# Autodesk Inventor assembly: Ender 3 Pro Assembly
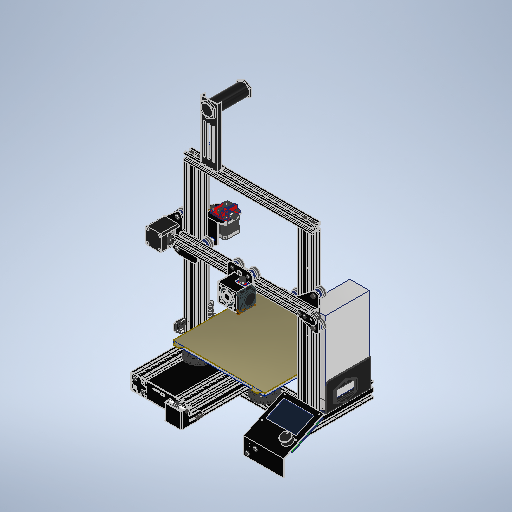
[picture p0: Inventor's stored thumbnail of the model, 512x512]
Saved by Autodesk Inventor 2025 (Build 290162000, 162)
## iProperties
Created: 2025-04-09
Part Number: Ender 3 Pro Assembly
Document SubType Name: Assembly
Designer: MAL16204
Author: MAL16204
## Documents named in this file (89)
- C:\Users\MAL16204\OneDrive - Pennsylvania Western University\Spring 2025\MECH 2400\CAD Projects\Final Project\Ender 3 Pro Assembly.iam
- C:\Users\MAL16204\OneDrive - Pennsylvania Western University\Spring 2025\MECH 2400\CAD Projects\Final Project\Aluminum Extrusions\4040 Central Profile.ipt
- C:\Users\MAL16204\OneDrive - Pennsylvania Western University\Spring 2025\MECH 2400\CAD Projects\Final Project\Aluminum Extrusions\4040 Left Profile.ipt
- C:\Users\MAL16204\OneDrive - Pennsylvania Western University\Spring 2025\MECH 2400\CAD Projects\Final Project\Aluminum Extrusions\4040 Right Profile.ipt
- C:\Users\MAL16204\OneDrive - Pennsylvania Western University\Spring 2025\MECH 2400\CAD Projects\Final Project\Aluminum Extrusions\2040 Right Profile.ipt
- C:\Users\MAL16204\OneDrive - Pennsylvania Western University\Spring 2025\MECH 2400\CAD Projects\Final Project\Aluminum Extrusions\2040 Left Profile.ipt
- C:\Users\MAL16204\OneDrive - Pennsylvania Western University\Spring 2025\MECH 2400\CAD Projects\Final Project\Aluminum Extrusions\2020 Top Profile.ipt
- C:\Users\MAL16204\OneDrive - Pennsylvania Western University\Spring 2025\MECH 2400\CAD Projects\Final Project\Miscellaneous Hardware\BS EN ISO 4762 - M5 x 50(1).ipt
- C:\Users\MAL16204\OneDrive - Pennsylvania Western University\Spring 2025\MECH 2400\CAD Projects\Final Project\Filament Holder\Support Frame (Filament Holder.ipt
- C:\Users\MAL16204\OneDrive - Pennsylvania Western University\Spring 2025\MECH 2400\CAD Projects\Final Project\Filament Holder\Support Tube (Filament Holder.ipt
- C:\Users\MAL16204\OneDrive - Pennsylvania Western University\Spring 2025\MECH 2400\CAD Projects\Final Project\Filament Holder\M30 Plastic Nut.ipt
- C:\Users\MAL16204\OneDrive - Pennsylvania Western University\Spring 2025\MECH 2400\CAD Projects\Final Project\Aluminum Extrusions\2020 X Profile.ipt
- C:\Users\MAL16204\OneDrive - Pennsylvania Western University\Spring 2025\MECH 2400\CAD Projects\Final Project\X-Axis Supporting Cast\X Adjustment Block.ipt
- C:\Users\MAL16204\OneDrive - Pennsylvania Western University\Spring 2025\MECH 2400\CAD Projects\Final Project\X-Axis Supporting Cast\X Motor Bracket.ipt
- C:\Users\MAL16204\OneDrive - Pennsylvania Western University\Spring 2025\MECH 2400\CAD Projects\Final Project\Stepper Motor 42mm\Assembly1.iam
- C:\Users\MAL16204\OneDrive - Pennsylvania Western University\Spring 2025\MECH 2400\CAD Projects\Final Project\Miscellaneous Hardware\Spacers for Rollers.ipt
- C:\Users\MAL16204\OneDrive - Pennsylvania Western University\Spring 2025\MECH 2400\CAD Projects\Final Project\Miscellaneous Hardware\Wheel_24.4mm v1\Wheel_24.4mm v1.ipt
- C:\Users\MAL16204\OneDrive - Pennsylvania Western University\Spring 2025\MECH 2400\CAD Projects\Final Project\Extruder\E Motor Bracket.ipt
- C:\Users\MAL16204\OneDrive - Pennsylvania Western University\Spring 2025\MECH 2400\CAD Projects\Final Project\LCD Support\LCD Support.ipt
- C:\Users\MAL16204\OneDrive - Pennsylvania Western University\Spring 2025\MECH 2400\CAD Projects\Final Project\LCD Support\LCD Knob.ipt
- C:\Users\MAL16204\OneDrive - Pennsylvania Western University\Spring 2025\MECH 2400\CAD Projects\Final Project\Aluminum Extrusions\4040 Y Profile.ipt
- C:\Users\MAL16204\OneDrive - Pennsylvania Western University\Spring 2025\MECH 2400\CAD Projects\Final Project\Z-Axis Supporting Cast\Z Stent.ipt
- C:\Users\MAL16204\OneDrive - Pennsylvania Western University\Spring 2025\MECH 2400\CAD Projects\Final Project\Hotend Assembly\Workspaces\Workspace\Extruder Plate.ipt
- C:\Users\MAL16204\OneDrive - Pennsylvania Western University\Spring 2025\MECH 2400\CAD Projects\Final Project\Hotend Assembly\Workspaces\Workspace\Hotend.ipt
- C:\Users\MAL16204\OneDrive - Pennsylvania Western University\Spring 2025\MECH 2400\CAD Projects\Final Project\Hotend Assembly\Workspaces\Workspace\Nozzle 0.4mm.ipt
- C:\Users\MAL16204\OneDrive - Pennsylvania Western University\Spring 2025\MECH 2400\CAD Projects\Final Project\Hotend Assembly\Workspaces\Workspace\Fan Cover.ipt
- C:\Users\MAL16204\OneDrive - Pennsylvania Western University\Spring 2025\MECH 2400\CAD Projects\Final Project\Y-Axis Supporting Cast\Y plate(GITHUB CR)\Y plate(GITHUB CR)\Y plate(GITHUB CR).ipt
- C:\Users\MAL16204\OneDrive - Pennsylvania Western University\Spring 2025\MECH 2400\CAD Projects\Final Project\Y-Axis Supporting Cast\Build Plate.ipt
- C:\Users\MAL16204\OneDrive - Pennsylvania Western University\Spring 2025\MECH 2400\CAD Projects\Final Project\Y-Axis Supporting Cast\Build Plate Rubber Supports.ipt
- C:\Users\MAL16204\OneDrive - Pennsylvania Western University\Spring 2025\MECH 2400\CAD Projects\Final Project\Z-Axis Supporting Cast\Z Nut.ipt
- C:\Users\MAL16204\OneDrive - Pennsylvania Western University\Spring 2025\MECH 2400\CAD Projects\Final Project\Sheetmetal Enclosures\Sheetmetal Enclosure Top.ipt
- C:\Users\MAL16204\OneDrive - Pennsylvania Western University\Spring 2025\MECH 2400\CAD Projects\Final Project\Sheetmetal Enclosures\Sheetmetal Enclosure Bottom.ipt
- C:\Users\MAL16204\OneDrive - Pennsylvania Western University\Spring 2025\MECH 2400\CAD Projects\Final Project\Y-Axis Supporting Cast\PEI Sheet (Build Plate).ipt
- C:\Users\MAL16204\OneDrive - Pennsylvania Western University\Spring 2025\MECH 2400\CAD Projects\Final Project\Y-Axis Supporting Cast\Hand Twisted Nut\Hand Twisted Nut\Hand Twisted Nut.ipt
- C:\Users\MAL16204\OneDrive - Pennsylvania Western University\Spring 2025\MECH 2400\CAD Projects\Final Project\Z-Axis Supporting Cast\Z Axis Motor Mount.ipt
- C:\Users\MAL16204\OneDrive - Pennsylvania Western University\Spring 2025\MECH 2400\CAD Projects\Final Project\Z-Axis Supporting Cast\Lead Screw Holder.ipt
- C:\Users\MAL16204\OneDrive - Pennsylvania Western University\Spring 2025\MECH 2400\CAD Projects\Final Project\Extruder\E housing\E housing.ipt
- C:\Users\MAL16204\OneDrive - Pennsylvania Western University\Spring 2025\MECH 2400\CAD Projects\Final Project\Extruder\E gear\E gear.ipt
- C:\Users\MAL16204\OneDrive - Pennsylvania Western University\Spring 2025\MECH 2400\CAD Projects\Final Project\Extruder\E idler tensioner\E idler tensioner.ipt
- C:\Users\MAL16204\OneDrive - Pennsylvania Western University\Spring 2025\MECH 2400\CAD Projects\Final Project\Z-Axis Supporting Cast\Lead Screw.ipt
- C:\Users\MAL16204\OneDrive - Pennsylvania Western University\Spring 2025\MECH 2400\CAD Projects\Final Project\LCD Support\lcd\lcd\lcd.ipt
- C:\Users\MAL16204\OneDrive - Pennsylvania Western University\Spring 2025\MECH 2400\CAD Projects\Final Project\Extruder\Extrusion Spring\Extrusion Spring\Extrusion Spring.ipt
- C:\Users\MAL16204\OneDrive - Pennsylvania Western University\Spring 2025\MECH 2400\CAD Projects\Final Project\Extruder\Pneumatic joint\Pneumatic joint\Pneumatic joint.ipt
- C:\Users\MAL16204\OneDrive - Pennsylvania Western University\Spring 2025\MECH 2400\CAD Projects\Final Project\Content Center Files\en-US\en-US\ISO 7380-1\ISO 7380-1 - M5 x 35.ipt
- C:\Users\MAL16204\OneDrive - Pennsylvania Western University\Spring 2025\MECH 2400\CAD Projects\Final Project\Content Center Files\en-US\en-US\ISO 7380-1\ISO 7380-1 - M5 x 25.ipt
- C:\Users\MAL16204\OneDrive - Pennsylvania Western University\Spring 2025\MECH 2400\CAD Projects\Final Project\Content Center Files\en-US\en-US\ISO 7380-1\ISO 7380-1 - M4 x 25.ipt
- C:\Users\MAL16204\OneDrive - Pennsylvania Western University\Spring 2025\MECH 2400\CAD Projects\Final Project\Power Supply\Power holder\Power holder\Power holder.ipt
- C:\Users\MAL16204\OneDrive - Pennsylvania Western University\Spring 2025\MECH 2400\CAD Projects\Final Project\Power Supply\24V15A power supply\24V15A power supply\24V15A power supply.ipt
- C:\Users\MAL16204\OneDrive - Pennsylvania Western University\Spring 2025\MECH 2400\CAD Projects\Final Project\Content Center Files\en-US\ISO 7380-1\ISO 7380-1 - M5 x 8.ipt
- C:\Users\MAL16204\OneDrive - Pennsylvania Western University\Spring 2025\MECH 2400\CAD Projects\Final Project\Content Center Files\en-US\ISO 7380-1\ISO 7380-1 - M4 x 6.ipt
- C:\Users\MAL16204\OneDrive - Pennsylvania Western University\Spring 2025\MECH 2400\CAD Projects\Final Project\Content Center Files\en-US\ISO 7380-1\ISO 7380-1 - M3 x 6.ipt
- C:\Users\MAL16204\OneDrive - Pennsylvania Western University\Spring 2025\MECH 2400\CAD Projects\Final Project\Content Center Files\en-US\BS EN ISO 4762\BS EN ISO 4762 - M2.5 x 4(1).ipt
- C:\Users\MAL16204\OneDrive - Pennsylvania Western University\Spring 2025\MECH 2400\CAD Projects\Final Project\Content Center Files\en-US\BS 4168(8)\BS 4168 - M4 x 25(7).ipt
- C:\Users\MAL16204\OneDrive - Pennsylvania Western University\Spring 2025\MECH 2400\CAD Projects\Final Project\Content Center Files\en-US\BS 4168(8)\BS 4168 - M3 x 16(7).ipt
- C:\Users\MAL16204\OneDrive - Pennsylvania Western University\Spring 2025\MECH 2400\CAD Projects\Final Project\Content Center Files\en-US\ISO 7380-1\ISO 7380-1 - M3 x 10.ipt
- C:\Users\MAL16204\OneDrive - Pennsylvania Western University\Spring 2025\MECH 2400\CAD Projects\Final Project\Content Center Files\en-US\ISO 4032(2)\ISO 4032 - M4 - ISO.ipt
- C:\Users\MAL16204\OneDrive - Pennsylvania Western University\Spring 2025\MECH 2400\CAD Projects\Final Project\Content Center Files\en-US\ISO 4032(2)\ISO 4032 - M5 - ISO.ipt
- C:\Users\MAL16204\OneDrive - Pennsylvania Western University\Spring 2025\MECH 2400\CAD Projects\Final Project\Miscellaneous Hardware\TSlot Nut.ipt
- C:\Users\MAL16204\OneDrive - Pennsylvania Western University\Spring 2025\MECH 2400\CAD Projects\Final Project\Content Center Files\en-US\ISO 7380-1\ISO 7380-1 - M5 x 10.ipt
- C:\Users\MAL16204\OneDrive - Pennsylvania Western University\Spring 2025\MECH 2400\CAD Projects\Final Project\Content Center Files\en-US\ISO 7380-1\ISO 7380-1 - M4 x 8.ipt
- C:\Users\MAL16204\OneDrive - Pennsylvania Western University\Spring 2025\MECH 2400\CAD Projects\Final Project\Content Center Files\en-US\ISO 7380-1\ISO 7380-1 - M5 x 12.ipt
- C:\Users\MAL16204\OneDrive - Pennsylvania Western University\Spring 2025\MECH 2400\CAD Projects\Final Project\Content Center Files\en-US\ISO 7380-1\ISO 7380-1 - M4 x 16.ipt
- C:\Users\MAL16204\OneDrive - Pennsylvania Western University\Spring 2025\MECH 2400\CAD Projects\Final Project\Content Center Files\en-US\BS EN ISO 4762\BS EN ISO 4762 - M3 x 12(1).ipt
- C:\Users\MAL16204\OneDrive - Pennsylvania Western University\Spring 2025\MECH 2400\CAD Projects\Final Project\Y-Axis Supporting Cast\Y Belt Adjuster.ipt
- C:\Users\MAL16204\OneDrive - Pennsylvania Western University\Spring 2025\MECH 2400\CAD Projects\Final Project\Y-Axis Supporting Cast\Roller Spacers.ipt
- C:\Users\MAL16204\OneDrive - Pennsylvania Western University\Spring 2025\MECH 2400\CAD Projects\Final Project\Y-Axis Supporting Cast\Belt Tension Rollers.ipt
- C:\Users\MAL16204\OneDrive - Pennsylvania Western University\Spring 2025\MECH 2400\CAD Projects\Final Project\Content Center Files\en-US\ISO 4762(2)\ISO 4762 - M3 x 30ISO.ipt
- C:\Users\MAL16204\OneDrive - Pennsylvania Western University\Spring 2025\MECH 2400\CAD Projects\Final Project\Content Center Files\en-US\ISO 4032(2)\ISO 4032 - M3.5 - ISO.ipt
- C:\Users\MAL16204\OneDrive - Pennsylvania Western University\Spring 2025\MECH 2400\CAD Projects\Final Project\Content Center Files\en-US\BS EN ISO 4762\BS EN ISO 4762 - M4 x 40(1).ipt
- C:\Users\MAL16204\OneDrive - Pennsylvania Western University\Spring 2025\MECH 2400\CAD Projects\Final Project\Content Center Files\en-US\ISO 7380-1\ISO 7380-1 - M3 x 16.ipt
- C:\Users\MAL16204\OneDrive - Pennsylvania Western University\Spring 2025\MECH 2400\CAD Projects\Final Project\Hotend Assembly\Nozzle fan\Nozzle fan\Nozzle fan.ipt
- C:\Users\MAL16204\OneDrive - Pennsylvania Western University\Spring 2025\MECH 2400\CAD Projects\Final Project\Content Center Files\en-US\BS EN ISO 4762\BS EN ISO 4762 - M3 x 8(1).ipt
- C:\Users\MAL16204\OneDrive - Pennsylvania Western University\Spring 2025\MECH 2400\CAD Projects\Final Project\Hotend Assembly\Nozzle fan duct\Nozzle fan duct\Nozzle fan duct.ipt
- C:\Users\MAL16204\OneDrive - Pennsylvania Western University\Spring 2025\MECH 2400\CAD Projects\Final Project\Hotend Assembly\Cold section fan\Cold section fan\Cold section fan.ipt
- C:\Users\MAL16204\OneDrive - Pennsylvania Western University\Spring 2025\MECH 2400\CAD Projects\Final Project\Y-Axis Supporting Cast\Y Motor Bracket.ipt
- C:\Users\MAL16204\OneDrive - Pennsylvania Western University\Spring 2025\MECH 2400\CAD Projects\Final Project\Y-Axis Supporting Cast\Y Limit Switch Bracket.ipt
- C:\Users\MAL16204\OneDrive - Pennsylvania Western University\Spring 2025\MECH 2400\CAD Projects\Final Project\Y-Axis Supporting Cast\limit switch\limit switch\limit switch.ipt
- C:\Users\MAL16204\OneDrive - Pennsylvania Western University\Spring 2025\MECH 2400\CAD Projects\Final Project\Content Center Files\en-US\ISO 7380-1\ISO 7380-1 - M4 x 10.ipt
- C:\Users\MAL16204\OneDrive - Pennsylvania Western University\Spring 2025\MECH 2400\CAD Projects\Final Project\Z-Axis Supporting Cast\Z Limit Switch Bracket.ipt
- C:\Users\MAL16204\OneDrive - Pennsylvania Western University\Spring 2025\MECH 2400\CAD Projects\Final Project\Content Center Files\en-US\ISO 7380-1\ISO 7380-1 - M4 x 30.ipt
- C:\Users\MAL16204\OneDrive - Pennsylvania Western University\Spring 2025\MECH 2400\CAD Projects\Final Project\Miscellaneous Hardware\Eccentric Column.ipt
- C:\Users\MAL16204\OneDrive - Pennsylvania Western University\Spring 2025\MECH 2400\CAD Projects\Final Project\Content Center Files\en-US\ISO 10642(1)\ISO 10642 - M3 x  20.ipt
- C:\Users\MAL16204\OneDrive - Pennsylvania Western University\Spring 2025\MECH 2400\CAD Projects\Final Project\Content Center Files\en-US\ISO 4026\ISO 4026 - M3 x 5 - ISO.ipt
- C:\Users\MAL16204\OneDrive - Pennsylvania Western University\Spring 2025\MECH 2400\CAD Projects\Final Project\Content Center Files\en-US\ISO 104\ISO 104 - 0 70 - 4 x 12 x 4.ipt
- C:\Users\MAL16204\OneDrive - Pennsylvania Western University\Spring 2025\MECH 2400\CAD Projects\Final Project\Content Center Files\en-US\BS EN ISO 4762\BS EN ISO 4762 - M3 x 6(1).ipt
- C:\Users\MAL16204\OneDrive - Pennsylvania Western University\Spring 2025\MECH 2400\CAD Projects\Final Project\X-Axis Supporting Cast\XEndStopHolder.ipt
- C:\Users\MAL16204\OneDrive - Pennsylvania Western University\Spring 2025\MECH 2400\CAD Projects\Final Project\Content Center Files\en-US\BS EN ISO 4762\BS EN ISO 4762 - M4 x 25(1).ipt
- C:\Users\MAL16204\OneDrive - Pennsylvania Western University\Spring 2025\MECH 2400\CAD Projects\Final Project\Content Center Files\en-US\ISO 4762(2)\ISO 4762 - M2 x 3ISO.ipt
- C:\Users\MAL16204\OneDrive - Pennsylvania Western University\Spring 2025\MECH 2400\CAD Projects\Final Project\Content Center Files\en-US\ISO 7380-1\ISO 7380-1 - M3 x 8.ipt
## Components (217 placed, 88 different names)
1. 4040 Central Profile:1 — Flush:1, Mate:1, Mate:2, Flush:2, Mate:3, Mate:4, Flush:4, Mate:21, Mate:22, Flush:11, Mate:39
2. 4040 Left Profile:1 — Flush:1, Mate:1, Mate:2, Mate:8, Flush:3, Rigid:2, Rigid:3, Rigid:4, Rigid:5, Mate:38, Flush:35, Flush:39, Mate:52, Mate:172
3. 4040 Right Profile:1 — Flush:2, Mate:3, Mate:4, Mate:5, Mate:6, Mate:7, Rigid:1, Cylindrical:1, Rigid:6, Rotational:1, Rigid:20, Mate:87, Flush:46
4. 2040 Right Profile:1 — Mate:5, Mate:6, Mate:7, Flush:5, Mate:24, Mate:25, Mate:26, Mate:88
5. 2040 Left Profile:1 — Mate:8, Flush:3, Flush:4, Mate:9, Flush:6, Flush:9, Mate:13, Mate:47, Mate:48, Mate:49, Mate:50, Mate:171, Flush:50, Mate:176, Mate:177, Mate:178, Mate:179
6. 2020 Top Profile:1 — Mate:9, Flush:5, Flush:6, Rigid:7, Rigid:8, Rigid:9, Rigid:10, Mate:10, Flush:7, Flush:8, Mate:115, Mate:116, Mate:118, Mate:119
7. BS EN ISO 4762 - Metric M5 x 50:1 — Rigid:1
8. BS EN ISO 4762 - Metric M5 x 50:2 — Cylindrical:1
9. BS EN ISO 4762 - Metric M5 x 50:3 — Rigid:3
10. BS EN ISO 4762 - Metric M5 x 50:4 — Rigid:2
11. BS EN ISO 4762 - Metric M5 x 50:5 — Rigid:5
12. BS EN ISO 4762 - Metric M5 x 50:6 — Rigid:4
13. BS EN ISO 4762 - Metric M5 x 50:7 — Rigid:6
14. BS EN ISO 4762 - Metric M5 x 50:8 — Rotational:1
15. BS EN ISO 4762 - Metric M5 x 50:9 — Rigid:8
16. BS EN ISO 4762 - Metric M5 x 50:10 — Rigid:7
17. BS EN ISO 4762 - Metric M5 x 50:11 — Rigid:9
18. BS EN ISO 4762 - Metric M5 x 50:12 — Rigid:10
19. Support Frame (Filament Holder:1 — Mate:10, Flush:7, Flush:8, Mate:117, Mate:120, Insert:27, Insert:28, Rigid:75
20. Support Tube (Filament Holder:1 — Rigid:11, Rigid:75, Rigid:76
21. M30 Plastic Nut:1 — Rigid:11
22. X Motor Bracket:1 — Mate:52, Rigid:61, Rigid:62, Mate:55, Mate:56, Mate:57, Rigid:63, Mate:71, Mate:72, Mate:73, Mate:74, Mate:81, Mate:82, Rigid:70, Insert:33, Insert:34, Mate:197, Mate:198, Mate:207
23. Spacers for Rollers:1 — Rotational:5, Rigid:62
24. Spacers for Rollers:2 — Rotational:3, Rigid:61
25. Spacers for Rollers:3 — Rotational:4, Rigid:63
26. Wheel_24.4mm v1:1 — Rotational:4, Rigid:16
27. Wheel_24.4mm v1:2 — Rotational:3, Rigid:17
28. Wheel_24.4mm v1:3 — Rotational:5, Flush:9, Mate:13, Rigid:15
29. E Motor Bracket:1 — Rigid:18, Rigid:19, Mate:35, Mate:36, Mate:37, Mate:58, Mate:59, Mate:64, Rotation/Translation:1, Mate:65, Mate:104, Mate:106, Mate:108, Mate:208, Mate:210
30. Spacers for Rollers:4 — Rigid:15, Rigid:19
31. Spacers for Rollers:5 — Rigid:16
32. Spacers for Rollers:6 — Rigid:17, Rigid:18
33. X Adjustment Block:1 — Mate:84, Flush:45, Mate:121, Mate:124, Mate:127, Insert:30, Insert:31, Mate:148, Mate:149
34. LCD Support:1 — Rigid:20, Rotational:6, Insert:6, Insert:7, Rigid:73
35. LCD Knob:1 — Rotational:6
36. 4040 Y Profile:1 — Mate:21, Mate:22, Flush:11, Rigid:21, Rigid:22, Rigid:23, Rigid:24, Flush:33, Flush:34, Mate:31, Mate:136, Flush:47, Mate:137, Mate:139, Mate:141, Mate:156, Mate:157, Mate:158, Mate:164, Mate:165, Mate:166, Mate:168, Mate:169, Flush:49
37. BS EN ISO 4762 - Metric M5 x 50:13 — Rigid:21
38. BS EN ISO 4762 - Metric M5 x 50:14 — Rigid:22
39. BS EN ISO 4762 - Metric M5 x 50:15 — Rigid:23
40. BS EN ISO 4762 - Metric M5 x 50:16 — Rigid:24
41. Z Stent:1 — Rigid:26, Rigid:27, Rigid:28, Flush:44, Mate:83, Rigid:72, Mate:110, Mate:112, Insert:29, Insert:32
42. Spacers for Rollers:8 — Rigid:26, Mate:28, Rigid:67
43. Spacers for Rollers:9 — Rigid:27, Mate:27
44. Spacers for Rollers:10 — Rigid:28, Mate:29
45. Wheel_24.4mm v1:4 — Mate:25, Mate:29, Mate:114
46. Wheel_24.4mm v1:5 — Mate:26, Mate:28, Rigid:67, Rigid:68
47. Wheel_24.4mm v1:6 — Mate:24, Mate:27, Rigid:69
48. Extruder Plate:1 — Rigid:29, Rigid:31, Rigid:35, Rigid:37, Insert:3, Insert:4, Flush:43, Rigid:82, Mate:190, Mate:192
49. Wheel_24.4mm v1:7 — Rigid:81, Rigid:84
50. Wheel_24.4mm v1:8 — Rigid:33, Mate:78, Mate:98
51. Wheel_24.4mm v1:9 — Rigid:34, Mate:77, Mate:100
52. Spacers for Rollers:11 — Rigid:29, Rigid:34
53. Spacers for Rollers:13 — Rigid:31, Rigid:33
54. Hotend:1 — Rigid:35, Rigid:36, Rigid:66, Mate:186, Mate:187, Mate:188, Mate:189, Flush:51
55. Nozzle 0.4mm:1 — Rigid:36
56. Fan Cover:1 — Rigid:37, Rigid:74, Mate:150, Mate:151, Mate:152, Mate:153, Mate:154, Mate:155, Mate:191, Mate:193, Mate:212, Mate:218, Mate:220, Mate:222
57. Spacers for Rollers:14 — Rigid:43, Rigid:46
58. Spacers for Rollers:15 — Rigid:44, Rigid:45
59. Wheel_24.4mm v1:12 — Rigid:43, Insert:57
60. Wheel_24.4mm v1:13 — Rigid:44, Flush:34, Insert:58
61. Y plate(GITHUB CR):1 — Rigid:45, Rigid:46, Flush:33, Mate:31, Mate:32, Mate:33, Mate:34, Mate:183, Mate:185, Rigid:78, Rigid:80
62. Wheel_24.4mm v1:15 — Rigid:77
63. Build Plate:1 — Rigid:51, Rigid:52, Rigid:53, Rigid:54, Mate:33, Mate:34, Mate:42, Flush:37, Flush:38, Rigid:56, Rigid:57, Rigid:58, Rigid:59
64. Build Plate Rubber Supports:1 — Rigid:51, Mate:32
65. Build Plate Rubber Supports:2 — Rigid:52
66. Build Plate Rubber Supports:3 — Rigid:54
67. Build Plate Rubber Supports:4 — Rigid:53
68. Assembly1:2 [sub-assembly] — Mate:35, Mate:36, Mate:37, Mate:60, Rotational:62
69. Sheetmetal Enclosure Top:1 — Mate:38, Mate:39, Flush:35, Mate:40, Mate:41, Flush:36, Insert:8, Insert:9
70. Sheetmetal Enclosure Bottom:1 — Mate:40, Mate:41, Flush:36, Insert:59, Insert:60
71. PEI Sheet (Build Plate):1 — Mate:42, Flush:37, Flush:38, Mate:80
72. Hand Twisted Nut:1 — Rigid:59
73. Hand Twisted Nut:2 — Rigid:56
74. Hand Twisted Nut:3 — Rigid:58
75. Hand Twisted Nut:4 — Rigid:57
76. Assembly1:3 [sub-assembly] — Mate:47, Flush:39, Mate:51, Rotational:61
77. Z Axis Motor Mount:1 — Mate:48, Mate:49, Mate:50, Mate:51, Mate:94, Mate:95, Insert:16, Insert:17
78. Lead Screw Holder:1 — Rotational:61, Rigid:64, Rotation/Translation:1, Insert:14, Insert:15
79. Assembly1:4 [sub-assembly] — Mate:55, Mate:56, Mate:57
80. E housing:1 — Mate:58, Mate:59, Mate:60, Rigid:65, Mate:68, Mate:69, Mate:70, Rigid:71, Mate:96, Insert:18, Insert:20
81. E gear:1 — Rotational:62
82. E idler tensioner:1 — Rigid:65, Insert:35, Insert:61
83. Lead Screw:1 — Rigid:64, Mate:63
84. Z Nut:1 — Mate:63, Mate:64, Mate:65, Mate:209, Mate:211
85. lcd:1 — Rigid:73, Insert:23, Insert:24, Insert:25, Insert:26
86. Extrusion Spring:1 — Mate:68, Mate:69, Mate:70
87. Pneumatic joint:2 — Rigid:66
88. ISO 7380-1 M5 x 35:1 — Mate:71, Mate:72, Mate:107
89. ISO 7380-1 M5 x 35:2 — Mate:73, Mate:74, Mate:105
90. ISO 7380-1 M4 x 25:1 — Insert:3, Mate:99
91. ISO 7380-1 M4 x 25:2 — Insert:4, Mate:97
92. 2020 X Profile:1 — Flush:43, Mate:77, Mate:78, Mate:80, Mate:81, Mate:82, Flush:44, Mate:83, Mate:84, Flush:45, Mate:121, Mate:122, Mate:123, Mate:125, Mate:126
93. ISO 7380-1 M5 x 25:4 — Rigid:68, Mate:109
94. ISO 7380-1 M5 x 25:5 — Rigid:69, Mate:111
95. ISO 7380-1 M5 x 35:3 — Rigid:70, Mate:103
96. Power holder:1 — Mate:87, Mate:88, Flush:46, Mate:89, Mate:90, Mate:91
97. 24V15A power supply:1 — Mate:89, Mate:90, Mate:91
98. Pneumatic joint:3 — Rigid:71
99. ISO 7380-1 M5 x 8:1 — Insert:6
100. ISO 7380-1 M5 x 8:2 — Insert:7
101. ISO 7380-1 M4 x 6:1 — Insert:8
102. ISO 7380-1 M4 x 6:2 — Insert:9
103. BS EN ISO 4762 - Metric M2.5 x 4:1 — Insert:14
104. BS EN ISO 4762 - Metric M2.5 x 4:2 — Insert:15
105. BS 4168 : Part 8 Hexagon socket countersunk and button head screws - Metric series - Metric M4 x 25:1 — Mate:94
106. BS 4168 : Part 8 Hexagon socket countersunk and button head screws - Metric series - Metric M4 x 25:2 — Mate:95
107. ISO 7380-1 M3 x 6:5 — Insert:16
108. ISO 7380-1 M3 x 6:6 — Insert:17
109. BS 4168 : Part 8 Hexagon socket countersunk and button head screws - Metric series - Metric M3 x 16:1 — Mate:96
110. ISO 7380-1 M3 x 6:7 — Insert:18
111. ISO 7380-1 M3 x 6:9 — Insert:20
112. ISO 7380-1 M4 x 25:3 — Rigid:72, Mate:113
113. ISO 7380-1 M3 x 10:1 — Insert:23
114. ISO 7380-1 M3 x 10:2 — Insert:24
115. ISO 7380-1 M3 x 10:3 — Insert:25
116. ISO 7380-1 M3 x 10:4 — Insert:26
117. ISO 4032 M4:1 — Mate:97, Mate:98
118. ISO 4032 M4:2 — Mate:99, Mate:100
119. ISO 4032 M5:2 — Mate:103, Mate:104
120. ISO 4032 M5:3 — Mate:105, Mate:106
121. ISO 4032 M5:4 — Mate:107, Mate:108
122. ISO 4032 M5:5 — Mate:109, Mate:110
123. ISO 4032 M5:6 — Mate:111, Mate:112
124. ISO 4032 M4:3 — Mate:113, Mate:114
125. TSlot Nut:1 — Mate:115, Mate:116, Mate:117
126. TSlot Nut:2 — Mate:118, Mate:119, Mate:120
127. ISO 7380-1 M5 x 8:3 — Insert:27
128. ISO 7380-1 M5 x 8:4 — Insert:28
129. ISO 7380-1 M5 x 10:1 — Insert:29
130. TSlot Nut:4 — Mate:122, Mate:123, Mate:124
131. TSlot Nut:5 — Mate:125, Mate:126, Mate:127
132. ISO 7380-1 M4 x 8:1 — Insert:30
133. ISO 7380-1 M4 x 8:2 — Insert:31
134. ISO 7380-1 M5 x 12:1 — Insert:32
135. ISO 7380-1 M4 x 16:1 — Insert:33
136. ISO 7380-1 M4 x 16:2 — Insert:34
137. BS EN ISO 4762 - Metric M3 x 12:1 — Insert:35
138. Y Belt Adjuster:1 — Mate:128, Mate:129, Mate:130, Mate:131, Insert:36, Insert:37, Mate:136, Flush:47, Mate:137, Mate:138, Mate:140, Mate:143, Mate:145
139. Roller Spacers:1 — Mate:128, Mate:129, Mate:134, Mate:135
140. Roller Spacers:2 — Mate:130, Mate:131
141. Belt Tension Rollers:1 — Mate:132, Mate:133, Mate:135
142. Belt Tension Rollers:2 — Mate:132, Mate:133, Mate:134
143. ISO 4762 M3 x 30:1 — Insert:36
144. ISO 4032 M3.5:1 — Insert:37
145. BS EN ISO 4762 - Metric M4 x 40:1 — Mate:138, Mate:139, Mate:144
146. BS EN ISO 4762 - Metric M4 x 40:2 — Mate:140, Mate:141, Mate:142
147. ISO 4032 M4:4 — Mate:142, Mate:143
148. ISO 4032 M4:5 — Mate:144, Mate:145
149. Belt Tension Rollers:3 — Mate:146, Mate:147, Mate:149, Insert:38
150. Belt Tension Rollers:4 — Mate:146, Mate:147, Mate:148
151. ISO 7380-1 M3 x 16:1 — Insert:38
152. Nozzle fan:1 — Rigid:74, Insert:39, Insert:40, Insert:41, Insert:42
153. BS EN ISO 4762 - Metric M3 x 8:1 — Insert:39
154. BS EN ISO 4762 - Metric M3 x 8:2 — Insert:40
155. BS EN ISO 4762 - Metric M3 x 8:3 — Insert:41
156. BS EN ISO 4762 - Metric M3 x 8:4 — Insert:42
157. Nozzle fan duct:1 — Mate:150, Mate:151, Mate:152, Mate:221, Mate:223
158. Cold section fan:1 — Mate:153, Mate:154, Mate:155, Mate:213, Mate:219
159. Y Motor Bracket:1 — Mate:156, Mate:157, Mate:158, Mate:159, Mate:160, Flush:48, Insert:65, Insert:66, Mate:225, Mate:227, Mate:229, Mate:231
160. Assembly1:5 [sub-assembly] — Mate:159, Mate:160, Flush:48, Mate:224, Mate:226, Mate:228, Mate:230
161. Y Limit Switch Bracket:1 — Mate:161, Mate:162, Mate:163, Mate:164, Mate:167, Mate:170, Flush:49, Insert:45, Insert:46
162. limit switch:1 — Insert:43, Insert:44, Mate:161
163. ISO 7380-1 M3 x 6:12 — Insert:43, Mate:163
164. ISO 7380-1 M3 x 6:13 — Insert:44, Mate:162
165. TSlot Nut:6 — Mate:165, Mate:166, Mate:167
166. TSlot Nut:7 — Mate:168, Mate:169, Mate:170
167. ISO 7380-1 M4 x 10:1 — Insert:45
168. ISO 7380-1 M4 x 10:2 — Insert:46
169. Z Limit Switch Bracket:1 — Mate:171, Mate:172, Mate:173, Mate:174, Mate:175, Flush:50, Mate:180, Mate:181, Insert:49, Insert:50
170. limit switch:2 — Mate:173, Mate:174, Mate:175, Insert:47, Insert:48
171. ISO 7380-1 M3 x 6:14 — Insert:47
172. ISO 7380-1 M3 x 6:15 — Insert:48
173. TSlot Nut:8 — Mate:176, Mate:177, Mate:181
174. TSlot Nut:9 — Mate:178, Mate:179, Mate:180
175. ISO 7380-1 M4 x 10:3 — Insert:49
176. ISO 7380-1 M4 x 10:4 — Insert:50
177. M30 Plastic Nut:2 — Rigid:76
178. ISO 7380-1 M4 x 30:3 — Insert:57, Mate:184
179. ISO 7380-1 M4 x 30:4 — Insert:58, Mate:182
180. ISO 4032 M4:6 — Mate:182, Mate:183
181. ISO 4032 M4:7 — Mate:184, Mate:185
182. Eccentric Column:1 — Rigid:77, Rigid:78
183. Wheel_24.4mm v1:16
184. Eccentric Column:2 — Rigid:80
185. Eccentric Column:3 — Rigid:81, Rigid:82, Rigid:83
186. ISO 7380-1 M4 x 25:4 — Rigid:83
187. ISO 4032 M4:8 — Rigid:84
188. ISO 10642 M3x20:1 — Mate:186
189. ISO 10642 M3x20:2 — Mate:187
190. ISO 4026 M3 x 5:1 — Mate:188, Flush:51
191. ISO 4026 M3 x 5:2 — Mate:189
192. ISO 7380-1 M3 x 6:16 — Mate:190, Mate:191
193. ISO 7380-1 M3 x 6:17 — Mate:192, Mate:193
194. ISO 7380-1 M3 x 6:18 — Insert:59
195. ISO 7380-1 M3 x 6:19 — Insert:60
196. ISO 104 (Single Direction) 0 70 - 4 x 12 x 4:1 — Insert:61, Insert:62
197. BS EN ISO 4762 - Metric M3 x 6:1 — Insert:62
198. XEndStopHolder:1 — Mate:194, Mate:195, Mate:196, Mate:197, Mate:198, Mate:199, Mate:200, Mate:201, Mate:202, Mate:203, Mate:204, Mate:205, Mate:206, Mate:207
199. limit switch:3 — Mate:194, Mate:195, Mate:196, Insert:63, Insert:64
200. ISO 7380-1 M3 x 6:20 — Insert:63
201. ISO 7380-1 M3 x 6:21 — Insert:64
202. BS EN ISO 4762 - Metric M4 x 25:1 — Mate:199, Mate:200
203. BS EN ISO 4762 - Metric M4 x 25:2 — Mate:201, Mate:202
204. BS EN ISO 4762 - Metric M4 x 25:3 — Mate:203, Mate:204
205. BS EN ISO 4762 - Metric M4 x 25:4 — Mate:205, Mate:206
206. ISO 7380-1 M3 x 6:22 — Mate:208, Mate:209
207. ISO 7380-1 M3 x 6:23 — Mate:210, Mate:211
208. ISO 4762 M2 x 3:1 — Mate:212, Mate:213
209. ISO 4762 M2 x 3:4 — Mate:218, Mate:219
210. ISO 4762 M2 x 3:5 — Mate:220, Mate:221
211. ISO 4762 M2 x 3:6 — Mate:222, Mate:223
212. ISO 7380-1 M3 x 16:2 — Insert:65
213. ISO 7380-1 M3 x 16:3 — Insert:66
214. ISO 7380-1 M3 x 8:1 — Mate:224, Mate:225
215. ISO 7380-1 M3 x 8:2 — Mate:226, Mate:227
216. ISO 7380-1 M3 x 8:3 — Mate:228, Mate:229
217. ISO 7380-1 M3 x 8:4 — Mate:230, Mate:231
## Relationships (349: Mate 197, WeldJoint 67, Insert 50, Flush 26, RevoluteJoint 7, CylindricalJoint 1, RelateRotateTranslate 1)
- Flush:1: 4040 Central Profile:1 ↔ 4040 Left Profile:1
- Mate:1: 4040 Central Profile:1 ↔ 4040 Left Profile:1
- Mate:2: 4040 Central Profile:1 ↔ 4040 Left Profile:1
- Flush:2: 4040 Central Profile:1 ↔ 4040 Right Profile:1
- Mate:3: 4040 Central Profile:1 ↔ 4040 Right Profile:1
- Mate:4: 4040 Central Profile:1 ↔ 4040 Right Profile:1
- Mate:5: 4040 Right Profile:1 ↔ 2040 Right Profile:1
- Mate:6: 4040 Right Profile:1 ↔ 2040 Right Profile:1
- Mate:7: 4040 Right Profile:1 ↔ 2040 Right Profile:1
- Mate:8: 4040 Left Profile:1 ↔ 2040 Left Profile:1
- Flush:3: 4040 Left Profile:1 ↔ 2040 Left Profile:1
- Flush:4 (-4.5 mm): 4040 Central Profile:1 ↔ 2040 Left Profile:1
- Mate:9: 2040 Left Profile:1 ↔ 2020 Top Profile:1
- Flush:5: 2040 Right Profile:1 ↔ 2020 Top Profile:1
- Flush:6: 2040 Left Profile:1 ↔ 2020 Top Profile:1
- Rigid:1 [WeldJoint]: 4040 Right Profile:1 ↔ BS EN ISO 4762 - Metric M5 x 50:1
- Cylindrical:1: 4040 Right Profile:1 ↔ BS EN ISO 4762 - Metric M5 x 50:2
- Rigid:2 [WeldJoint]: 4040 Left Profile:1 ↔ BS EN ISO 4762 - Metric M5 x 50:4
- Rigid:3 [WeldJoint]: 4040 Left Profile:1 ↔ BS EN ISO 4762 - Metric M5 x 50:3
- Rigid:4 [WeldJoint]: 4040 Left Profile:1 ↔ BS EN ISO 4762 - Metric M5 x 50:6
- Rigid:5 [WeldJoint]: 4040 Left Profile:1 ↔ BS EN ISO 4762 - Metric M5 x 50:5
- Rigid:6 [WeldJoint]: 4040 Right Profile:1 ↔ BS EN ISO 4762 - Metric M5 x 50:7
- Rotational:1 [RevoluteJoint]: 4040 Right Profile:1 ↔ BS EN ISO 4762 - Metric M5 x 50:8
- Rigid:7 [WeldJoint]: 2020 Top Profile:1 ↔ BS EN ISO 4762 - Metric M5 x 50:10
- Rigid:8 [WeldJoint]: 2020 Top Profile:1 ↔ BS EN ISO 4762 - Metric M5 x 50:9
- Rigid:9 [WeldJoint]: 2020 Top Profile:1 ↔ BS EN ISO 4762 - Metric M5 x 50:11
- Rigid:10 [WeldJoint]: 2020 Top Profile:1 ↔ BS EN ISO 4762 - Metric M5 x 50:12
- Mate:10: 2020 Top Profile:1 ↔ Support Frame (Filament Holder:1
- Flush:7: 2020 Top Profile:1 ↔ Support Frame (Filament Holder:1
- Flush:8 (45 mm): 2020 Top Profile:1 ↔ Support Frame (Filament Holder:1
- Rigid:11 [WeldJoint]: Support Tube (Filament Holder:1 ↔ M30 Plastic Nut:1
- Rotational:3 [RevoluteJoint]: Spacers for Rollers:2 ↔ Wheel_24.4mm v1:2
- Rotational:4 [RevoluteJoint]: Spacers for Rollers:3 ↔ Wheel_24.4mm v1:1
- Rotational:5 [RevoluteJoint]: Spacers for Rollers:1 ↔ Wheel_24.4mm v1:3
- Flush:9: 2040 Left Profile:1 ↔ Wheel_24.4mm v1:3
- Mate:13 (16 mm): 2040 Left Profile:1 ↔ Wheel_24.4mm v1:3
- Rigid:15 [WeldJoint]: Wheel_24.4mm v1:3 ↔ Spacers for Rollers:4
- Rigid:16 [WeldJoint]: Wheel_24.4mm v1:1 ↔ Spacers for Rollers:5
- Rigid:17 [WeldJoint]: Wheel_24.4mm v1:2 ↔ Spacers for Rollers:6
- Rigid:18 [WeldJoint]: E Motor Bracket:1 ↔ Spacers for Rollers:6
- Rigid:19 [WeldJoint]: E Motor Bracket:1 ↔ Spacers for Rollers:4
- Rigid:20 [WeldJoint]: 4040 Right Profile:1 ↔ LCD Support:1
- Rotational:6 [RevoluteJoint]: LCD Support:1 ↔ LCD Knob:1
- Mate:21: 4040 Central Profile:1 ↔ 4040 Y Profile:1
- Mate:22: 4040 Central Profile:1 ↔ 4040 Y Profile:1
- Flush:11 (-155 mm): 4040 Central Profile:1 ↔ 4040 Y Profile:1
- Rigid:21 [WeldJoint]: 4040 Y Profile:1 ↔ BS EN ISO 4762 - Metric M5 x 50:13
- Rigid:22 [WeldJoint]: 4040 Y Profile:1 ↔ BS EN ISO 4762 - Metric M5 x 50:14
- Rigid:23 [WeldJoint]: 4040 Y Profile:1 ↔ BS EN ISO 4762 - Metric M5 x 50:15
- Rigid:24 [WeldJoint]: 4040 Y Profile:1 ↔ BS EN ISO 4762 - Metric M5 x 50:16
- Rigid:26 [WeldJoint]: Z Stent:1 ↔ Spacers for Rollers:8
- Rigid:27 [WeldJoint]: Z Stent:1 ↔ Spacers for Rollers:9
- Rigid:28 [WeldJoint]: Z Stent:1 ↔ Spacers for Rollers:10
- Mate:24: 2040 Right Profile:1 ↔ Wheel_24.4mm v1:6
- Mate:25: 2040 Right Profile:1 ↔ Wheel_24.4mm v1:4
- Mate:26: 2040 Right Profile:1 ↔ Wheel_24.4mm v1:5
- Mate:27: Spacers for Rollers:9 ↔ Wheel_24.4mm v1:6
- Mate:28: Spacers for Rollers:8 ↔ Wheel_24.4mm v1:5
- Mate:29: Spacers for Rollers:10 ↔ Wheel_24.4mm v1:4
- Rigid:29 [WeldJoint]: Extruder Plate:1 ↔ Spacers for Rollers:11
- Rigid:31 [WeldJoint]: Extruder Plate:1 ↔ Spacers for Rollers:13
- Rigid:33 [WeldJoint]: Wheel_24.4mm v1:8 ↔ Spacers for Rollers:13
- Rigid:34 [WeldJoint]: Wheel_24.4mm v1:9 ↔ Spacers for Rollers:11
- Rigid:35 [WeldJoint]: Extruder Plate:1 ↔ Hotend:1
- Rigid:36 [WeldJoint]: Hotend:1 ↔ Nozzle 0.4mm:1
- Rigid:37 [WeldJoint]: Extruder Plate:1 ↔ Fan Cover:1
- Rigid:43 [WeldJoint]: Spacers for Rollers:14 ↔ Wheel_24.4mm v1:12
- Rigid:44 [WeldJoint]: Spacers for Rollers:15 ↔ Wheel_24.4mm v1:13
- Rigid:45 [WeldJoint]: Spacers for Rollers:15 ↔ Y plate(GITHUB CR):1
- Rigid:46 [WeldJoint]: Spacers for Rollers:14 ↔ Y plate(GITHUB CR):1
- Flush:33: 4040 Y Profile:1 ↔ Y plate(GITHUB CR):1
- Flush:34 (10 mm): 4040 Y Profile:1 ↔ Wheel_24.4mm v1:13
- Mate:31: 4040 Y Profile:1 ↔ Y plate(GITHUB CR):1
- Rigid:51 [WeldJoint]: Build Plate:1 ↔ Build Plate Rubber Supports:1
- Rigid:52 [WeldJoint]: Build Plate:1 ↔ Build Plate Rubber Supports:2
- Rigid:53 [WeldJoint]: Build Plate:1 ↔ Build Plate Rubber Supports:4
- Rigid:54 [WeldJoint]: Build Plate:1 ↔ Build Plate Rubber Supports:3
- Mate:32: Y plate(GITHUB CR):1 ↔ Build Plate Rubber Supports:1
- Mate:33: Y plate(GITHUB CR):1 ↔ Build Plate:1
- Mate:34: Y plate(GITHUB CR):1 ↔ Build Plate:1
- Mate:35: E Motor Bracket:1 ↔ Assembly1:2
- Mate:36: E Motor Bracket:1 ↔ Assembly1:2
- Mate:37: E Motor Bracket:1 ↔ Assembly1:2
- Mate:38: 4040 Left Profile:1 ↔ Sheetmetal Enclosure Top:1
- Mate:39: 4040 Central Profile:1 ↔ Sheetmetal Enclosure Top:1
- Flush:35: 4040 Left Profile:1 ↔ Sheetmetal Enclosure Top:1
- Mate:40 (0.8 mm): Sheetmetal Enclosure Top:1 ↔ Sheetmetal Enclosure Bottom:1
- Mate:41: Sheetmetal Enclosure Top:1 ↔ Sheetmetal Enclosure Bottom:1
- Flush:36: Sheetmetal Enclosure Top:1 ↔ Sheetmetal Enclosure Bottom:1
- Mate:42: Build Plate:1 ↔ PEI Sheet (Build Plate):1
- Flush:37: Build Plate:1 ↔ PEI Sheet (Build Plate):1
- Flush:38: Build Plate:1 ↔ PEI Sheet (Build Plate):1
- Rigid:56 [WeldJoint]: Build Plate:1 ↔ Hand Twisted Nut:2
- Rigid:57 [WeldJoint]: Build Plate:1 ↔ Hand Twisted Nut:4
- Rigid:58 [WeldJoint]: Build Plate:1 ↔ Hand Twisted Nut:3
- Rigid:59 [WeldJoint]: Build Plate:1 ↔ Hand Twisted Nut:1
- Mate:47: 2040 Left Profile:1 ↔ Assembly1:3
- Flush:39: 4040 Left Profile:1 ↔ Assembly1:3
- Mate:48: 2040 Left Profile:1 ↔ Z Axis Motor Mount:1
- Mate:49: 2040 Left Profile:1 ↔ Z Axis Motor Mount:1
- Mate:50: 2040 Left Profile:1 ↔ Z Axis Motor Mount:1
- Mate:51: Assembly1:3 ↔ Z Axis Motor Mount:1
- Rotational:61 [RevoluteJoint]: Assembly1:3 ↔ Lead Screw Holder:1
- Mate:52: 4040 Left Profile:1 ↔ X Motor Bracket:1
- Rigid:61 [WeldJoint]: X Motor Bracket:1 ↔ Spacers for Rollers:2
- Rigid:62 [WeldJoint]: X Motor Bracket:1 ↔ Spacers for Rollers:1
- Mate:55: X Motor Bracket:1 ↔ Assembly1:4
- Mate:56: X Motor Bracket:1 ↔ Assembly1:4
- Mate:57: X Motor Bracket:1 ↔ Assembly1:4
- Rigid:63 [WeldJoint]: X Motor Bracket:1 ↔ Spacers for Rollers:3
- Mate:58: E Motor Bracket:1 ↔ E housing:1
- Mate:59: E Motor Bracket:1 ↔ E housing:1
- Mate:60: Assembly1:2 ↔ E housing:1
- Rotational:62 [RevoluteJoint]: Assembly1:2 ↔ E gear:1
- Rigid:64 [WeldJoint]: Lead Screw Holder:1 ↔ Lead Screw:1
- Mate:63: Lead Screw:1 ↔ Z Nut:1
- Mate:64: E Motor Bracket:1 ↔ Z Nut:1
- Rotation/Translation:1 [RelateRotateTranslate] (20 mm): E Motor Bracket:1 ↔ Lead Screw Holder:1
- Mate:65 (1.5 mm): E Motor Bracket:1 ↔ Z Nut:1
- Rigid:65 [WeldJoint]: E housing:1 ↔ E idler tensioner:1
- Mate:68 (4 mm): E housing:1 ↔ Extrusion Spring:1
- Mate:69: E housing:1 ↔ Extrusion Spring:1
- Mate:70 (-2 mm): E housing:1 ↔ Extrusion Spring:1
- Rigid:66 [WeldJoint]: Hotend:1 ↔ Pneumatic joint:2
- Mate:71: X Motor Bracket:1 ↔ ISO 7380-1 M5 x 35:1
- Mate:72: X Motor Bracket:1 ↔ ISO 7380-1 M5 x 35:1
- Mate:73: X Motor Bracket:1 ↔ ISO 7380-1 M5 x 35:2
- Mate:74: X Motor Bracket:1 ↔ ISO 7380-1 M5 x 35:2
- Insert:3: Extruder Plate:1 ↔ ISO 7380-1 M4 x 25:1
- Insert:4: Extruder Plate:1 ↔ ISO 7380-1 M4 x 25:2
- Flush:43: Extruder Plate:1 ↔ 2020 X Profile:1
- Mate:77: Wheel_24.4mm v1:9 ↔ 2020 X Profile:1
- Mate:78 (15 mm): Wheel_24.4mm v1:8 ↔ 2020 X Profile:1
- Rigid:67 [WeldJoint]: Spacers for Rollers:8 ↔ Wheel_24.4mm v1:5
- Mate:80: PEI Sheet (Build Plate):1 ↔ 2020 X Profile:1
- Mate:81: X Motor Bracket:1 ↔ 2020 X Profile:1
- Mate:82: X Motor Bracket:1 ↔ 2020 X Profile:1
- Flush:44: Z Stent:1 ↔ 2020 X Profile:1
- Mate:83: Z Stent:1 ↔ 2020 X Profile:1
- Mate:84: X Adjustment Block:1 ↔ 2020 X Profile:1
- Flush:45: X Adjustment Block:1 ↔ 2020 X Profile:1
- Rigid:68 [WeldJoint]: Wheel_24.4mm v1:5 ↔ ISO 7380-1 M5 x 25:4
- Rigid:69 [WeldJoint]: Wheel_24.4mm v1:6 ↔ ISO 7380-1 M5 x 25:5
- Rigid:70 [WeldJoint]: X Motor Bracket:1 ↔ ISO 7380-1 M5 x 35:3
- Mate:87: 4040 Right Profile:1 ↔ Power holder:1
- Mate:88: 2040 Right Profile:1 ↔ Power holder:1
- Flush:46: 4040 Right Profile:1 ↔ Power holder:1
- Mate:89: Power holder:1 ↔ 24V15A power supply:1
- Mate:90: Power holder:1 ↔ 24V15A power supply:1
- Mate:91: Power holder:1 ↔ 24V15A power supply:1
- Rigid:71 [WeldJoint]: E housing:1 ↔ Pneumatic joint:3
- Insert:6: LCD Support:1 ↔ ISO 7380-1 M5 x 8:1
- Insert:7: LCD Support:1 ↔ ISO 7380-1 M5 x 8:2
- Insert:8: Sheetmetal Enclosure Top:1 ↔ ISO 7380-1 M4 x 6:1
- Insert:9: Sheetmetal Enclosure Top:1 ↔ ISO 7380-1 M4 x 6:2
- Insert:14: Lead Screw Holder:1 ↔ BS EN ISO 4762 - Metric M2.5 x 4:1
- Insert:15: Lead Screw Holder:1 ↔ BS EN ISO 4762 - Metric M2.5 x 4:2
- Mate:94: Z Axis Motor Mount:1 ↔ BS 4168 : Part 8 Hexagon socket countersunk and button head screws - Metric series - Metric M4 x 25:1
- Mate:95: Z Axis Motor Mount:1 ↔ BS 4168 : Part 8 Hexagon socket countersunk and button head screws - Metric series - Metric M4 x 25:2
- Insert:16: Z Axis Motor Mount:1 ↔ ISO 7380-1 M3 x 6:5
- Insert:17: Z Axis Motor Mount:1 ↔ ISO 7380-1 M3 x 6:6
- Mate:96: E housing:1 ↔ BS 4168 : Part 8 Hexagon socket countersunk and button head screws - Metric series - Metric M3 x 16:1
- Insert:18: E housing:1 ↔ ISO 7380-1 M3 x 6:7
- Insert:20: E housing:1 ↔ ISO 7380-1 M3 x 6:9
- Rigid:72 [WeldJoint]: Z Stent:1 ↔ ISO 7380-1 M4 x 25:3
- Rigid:73 [WeldJoint]: LCD Support:1 ↔ lcd:1
- Insert:23: lcd:1 ↔ ISO 7380-1 M3 x 10:1
- Insert:24: lcd:1 ↔ ISO 7380-1 M3 x 10:2
- Insert:25: lcd:1 ↔ ISO 7380-1 M3 x 10:3
- Insert:26: lcd:1 ↔ ISO 7380-1 M3 x 10:4
- Mate:97: ISO 7380-1 M4 x 25:2 ↔ ISO 4032 M4:1
- Mate:98: Wheel_24.4mm v1:8 ↔ ISO 4032 M4:1
- Mate:99: ISO 7380-1 M4 x 25:1 ↔ ISO 4032 M4:2
- Mate:100: Wheel_24.4mm v1:9 ↔ ISO 4032 M4:2
- Mate:103: ISO 7380-1 M5 x 35:3 ↔ ISO 4032 M5:2
- Mate:104: E Motor Bracket:1 ↔ ISO 4032 M5:2
- Mate:105: ISO 7380-1 M5 x 35:2 ↔ ISO 4032 M5:3
- Mate:106: E Motor Bracket:1 ↔ ISO 4032 M5:3
- Mate:107: ISO 7380-1 M5 x 35:1 ↔ ISO 4032 M5:4
- Mate:108: E Motor Bracket:1 ↔ ISO 4032 M5:4
- Mate:109: ISO 7380-1 M5 x 25:4 ↔ ISO 4032 M5:5
- Mate:110: Z Stent:1 ↔ ISO 4032 M5:5
- Mate:111: ISO 7380-1 M5 x 25:5 ↔ ISO 4032 M5:6
- Mate:112: Z Stent:1 ↔ ISO 4032 M5:6
- Mate:113: ISO 7380-1 M4 x 25:3 ↔ ISO 4032 M4:3
- Mate:114: Wheel_24.4mm v1:4 ↔ ISO 4032 M4:3
- Mate:115: 2020 Top Profile:1 ↔ TSlot Nut:1
- Mate:116: 2020 Top Profile:1 ↔ TSlot Nut:1
- Mate:117: Support Frame (Filament Holder:1 ↔ TSlot Nut:1
- Mate:118: 2020 Top Profile:1 ↔ TSlot Nut:2
- Mate:119: 2020 Top Profile:1 ↔ TSlot Nut:2
- Mate:120: Support Frame (Filament Holder:1 ↔ TSlot Nut:2
- Insert:27: Support Frame (Filament Holder:1 ↔ ISO 7380-1 M5 x 8:3
- Insert:28: Support Frame (Filament Holder:1 ↔ ISO 7380-1 M5 x 8:4
- Mate:121 (10 mm): X Adjustment Block:1 ↔ 2020 X Profile:1
- Insert:29: Z Stent:1 ↔ ISO 7380-1 M5 x 10:1
- Mate:122: 2020 X Profile:1 ↔ TSlot Nut:4
- Mate:123: 2020 X Profile:1 ↔ TSlot Nut:4
- Mate:124: X Adjustment Block:1 ↔ TSlot Nut:4
- Mate:125: 2020 X Profile:1 ↔ TSlot Nut:5
- Mate:126: 2020 X Profile:1 ↔ TSlot Nut:5
- Mate:127: X Adjustment Block:1 ↔ TSlot Nut:5
- Insert:30: X Adjustment Block:1 ↔ ISO 7380-1 M4 x 8:1
- Insert:31: X Adjustment Block:1 ↔ ISO 7380-1 M4 x 8:2
- Insert:32: Z Stent:1 ↔ ISO 7380-1 M5 x 12:1
- Insert:33: X Motor Bracket:1 ↔ ISO 7380-1 M4 x 16:1
- Insert:34: X Motor Bracket:1 ↔ ISO 7380-1 M4 x 16:2
- Insert:35: E idler tensioner:1 ↔ BS EN ISO 4762 - Metric M3 x 12:1
- Mate:128: Y Belt Adjuster:1 ↔ Roller Spacers:1
- Mate:129: Y Belt Adjuster:1 ↔ Roller Spacers:1
- Mate:130: Y Belt Adjuster:1 ↔ Roller Spacers:2
- Mate:131: Y Belt Adjuster:1 ↔ Roller Spacers:2
- Mate:132: Belt Tension Rollers:1 ↔ Belt Tension Rollers:2
- Mate:133: Belt Tension Rollers:1 ↔ Belt Tension Rollers:2
- Mate:134: Roller Spacers:1 ↔ Belt Tension Rollers:2
- Mate:135: Roller Spacers:1 ↔ Belt Tension Rollers:1
- Insert:36: Y Belt Adjuster:1 ↔ ISO 4762 M3 x 30:1
- Insert:37: Y Belt Adjuster:1 ↔ ISO 4032 M3.5:1
- Mate:136: 4040 Y Profile:1 ↔ Y Belt Adjuster:1
- Flush:47: 4040 Y Profile:1 ↔ Y Belt Adjuster:1
- Mate:137 (-25 mm): 4040 Y Profile:1 ↔ Y Belt Adjuster:1
- Mate:138: Y Belt Adjuster:1 ↔ BS EN ISO 4762 - Metric M4 x 40:1
- Mate:139: 4040 Y Profile:1 ↔ BS EN ISO 4762 - Metric M4 x 40:1
- Mate:140: Y Belt Adjuster:1 ↔ BS EN ISO 4762 - Metric M4 x 40:2
- Mate:141: 4040 Y Profile:1 ↔ BS EN ISO 4762 - Metric M4 x 40:2
- Mate:142: BS EN ISO 4762 - Metric M4 x 40:2 ↔ ISO 4032 M4:4
- Mate:143: Y Belt Adjuster:1 ↔ ISO 4032 M4:4
- Mate:144: BS EN ISO 4762 - Metric M4 x 40:1 ↔ ISO 4032 M4:5
- Mate:145: Y Belt Adjuster:1 ↔ ISO 4032 M4:5
- Mate:146: Belt Tension Rollers:3 ↔ Belt Tension Rollers:4
- Mate:147: Belt Tension Rollers:3 ↔ Belt Tension Rollers:4
- Mate:148: X Adjustment Block:1 ↔ Belt Tension Rollers:4
- Mate:149: X Adjustment Block:1 ↔ Belt Tension Rollers:3
- Insert:38: Belt Tension Rollers:3 ↔ ISO 7380-1 M3 x 16:1
- Rigid:74 [WeldJoint]: Fan Cover:1 ↔ Nozzle fan:1
- Insert:39: Nozzle fan:1 ↔ BS EN ISO 4762 - Metric M3 x 8:1
- Insert:40: Nozzle fan:1 ↔ BS EN ISO 4762 - Metric M3 x 8:2
- Insert:41: Nozzle fan:1 ↔ BS EN ISO 4762 - Metric M3 x 8:3
- Insert:42: Nozzle fan:1 ↔ BS EN ISO 4762 - Metric M3 x 8:4
- Mate:150: Fan Cover:1 ↔ Nozzle fan duct:1
- Mate:151: Fan Cover:1 ↔ Nozzle fan duct:1
- Mate:152: Fan Cover:1 ↔ Nozzle fan duct:1
- Mate:153: Fan Cover:1 ↔ Cold section fan:1
- Mate:154: Fan Cover:1 ↔ Cold section fan:1
- Mate:155: Fan Cover:1 ↔ Cold section fan:1
- Mate:156: 4040 Y Profile:1 ↔ Y Motor Bracket:1
- Mate:157 (-23 mm): 4040 Y Profile:1 ↔ Y Motor Bracket:1
- Mate:158: 4040 Y Profile:1 ↔ Y Motor Bracket:1
- Mate:159: Y Motor Bracket:1 ↔ Assembly1:5
- Mate:160: Y Motor Bracket:1 ↔ Assembly1:5
- Flush:48: Y Motor Bracket:1 ↔ Assembly1:5
- Insert:43: limit switch:1 ↔ ISO 7380-1 M3 x 6:12
- Insert:44: limit switch:1 ↔ ISO 7380-1 M3 x 6:13
- Mate:161: Y Limit Switch Bracket:1 ↔ limit switch:1
- Mate:162: Y Limit Switch Bracket:1 ↔ ISO 7380-1 M3 x 6:13
- Mate:163: Y Limit Switch Bracket:1 ↔ ISO 7380-1 M3 x 6:12
- Mate:164: 4040 Y Profile:1 ↔ Y Limit Switch Bracket:1
- Mate:165: 4040 Y Profile:1 ↔ TSlot Nut:6
- Mate:166: 4040 Y Profile:1 ↔ TSlot Nut:6
- Mate:167: Y Limit Switch Bracket:1 ↔ TSlot Nut:6
- Mate:168: 4040 Y Profile:1 ↔ TSlot Nut:7
- Mate:169: 4040 Y Profile:1 ↔ TSlot Nut:7
- Mate:170: Y Limit Switch Bracket:1 ↔ TSlot Nut:7
- Flush:49: 4040 Y Profile:1 ↔ Y Limit Switch Bracket:1
- Insert:45: Y Limit Switch Bracket:1 ↔ ISO 7380-1 M4 x 10:1
- Insert:46: Y Limit Switch Bracket:1 ↔ ISO 7380-1 M4 x 10:2
- Mate:171: 2040 Left Profile:1 ↔ Z Limit Switch Bracket:1
- Mate:172: 4040 Left Profile:1 ↔ Z Limit Switch Bracket:1
- Mate:173: Z Limit Switch Bracket:1 ↔ limit switch:2
- Mate:174: Z Limit Switch Bracket:1 ↔ limit switch:2
- Mate:175: Z Limit Switch Bracket:1 ↔ limit switch:2
- Flush:50: 2040 Left Profile:1 ↔ Z Limit Switch Bracket:1
- Insert:47: limit switch:2 ↔ ISO 7380-1 M3 x 6:14
- Insert:48: limit switch:2 ↔ ISO 7380-1 M3 x 6:15
- Mate:176: 2040 Left Profile:1 ↔ TSlot Nut:8
- Mate:177: 2040 Left Profile:1 ↔ TSlot Nut:8
- Mate:178: 2040 Left Profile:1 ↔ TSlot Nut:9
- Mate:179: 2040 Left Profile:1 ↔ TSlot Nut:9
- Mate:180: Z Limit Switch Bracket:1 ↔ TSlot Nut:9
- Mate:181: Z Limit Switch Bracket:1 ↔ TSlot Nut:8
- Insert:49: Z Limit Switch Bracket:1 ↔ ISO 7380-1 M4 x 10:3
- Insert:50: Z Limit Switch Bracket:1 ↔ ISO 7380-1 M4 x 10:4
- Rigid:75 [WeldJoint]: Support Frame (Filament Holder:1 ↔ Support Tube (Filament Holder:1
- Rigid:76 [WeldJoint] (-2 mm): Support Tube (Filament Holder:1 ↔ M30 Plastic Nut:2
- Insert:57: Wheel_24.4mm v1:12 ↔ ISO 7380-1 M4 x 30:3
- Insert:58: Wheel_24.4mm v1:13 ↔ ISO 7380-1 M4 x 30:4
- Mate:182: ISO 7380-1 M4 x 30:4 ↔ ISO 4032 M4:6
- Mate:183: Y plate(GITHUB CR):1 ↔ ISO 4032 M4:6
- Mate:184: ISO 7380-1 M4 x 30:3 ↔ ISO 4032 M4:7
- Mate:185: Y plate(GITHUB CR):1 ↔ ISO 4032 M4:7
- Rigid:77 [WeldJoint]: Wheel_24.4mm v1:15 ↔ Eccentric Column:1
- Rigid:78 [WeldJoint]: Y plate(GITHUB CR):1 ↔ Eccentric Column:1
- [WeldJoint]: Wheel_24.4mm v1:16 ↔ Eccentric Column:2
- Rigid:80 [WeldJoint]: Y plate(GITHUB CR):1 ↔ Eccentric Column:2
- Rigid:81 [WeldJoint]: Wheel_24.4mm v1:7 ↔ Eccentric Column:3
- Rigid:82 [WeldJoint]: Extruder Plate:1 ↔ Eccentric Column:3
- Rigid:83 [WeldJoint]: Eccentric Column:3 ↔ ISO 7380-1 M4 x 25:4
- Rigid:84 [WeldJoint]: Wheel_24.4mm v1:7 ↔ ISO 4032 M4:8
- Mate:186: Hotend:1 ↔ ISO 10642 M3x20:1
- Mate:187: Hotend:1 ↔ ISO 10642 M3x20:2
- Mate:188: Hotend:1 ↔ ISO 4026 M3 x 5:1
- Mate:189: Hotend:1 ↔ ISO 4026 M3 x 5:2
- Mate:190: Extruder Plate:1 ↔ ISO 7380-1 M3 x 6:16
- Mate:191: Fan Cover:1 ↔ ISO 7380-1 M3 x 6:16
- Mate:192: Extruder Plate:1 ↔ ISO 7380-1 M3 x 6:17
- Mate:193: Fan Cover:1 ↔ ISO 7380-1 M3 x 6:17
- Insert:59: Sheetmetal Enclosure Bottom:1 ↔ ISO 7380-1 M3 x 6:18
- Insert:60: Sheetmetal Enclosure Bottom:1 ↔ ISO 7380-1 M3 x 6:19
- Insert:61: E idler tensioner:1 ↔ ISO 104 (Single Direction) 0 70 - 4 x 12 x 4:1
- Insert:62: ISO 104 (Single Direction) 0 70 - 4 x 12 x 4:1 ↔ BS EN ISO 4762 - Metric M3 x 6:1
- Mate:194: XEndStopHolder:1 ↔ limit switch:3
- Mate:195: XEndStopHolder:1 ↔ limit switch:3
- Mate:196: XEndStopHolder:1 ↔ limit switch:3
- Insert:63: limit switch:3 ↔ ISO 7380-1 M3 x 6:20
- Insert:64: limit switch:3 ↔ ISO 7380-1 M3 x 6:21
- Mate:197: X Motor Bracket:1 ↔ XEndStopHolder:1
- Mate:198: X Motor Bracket:1 ↔ XEndStopHolder:1
- Mate:199: XEndStopHolder:1 ↔ BS EN ISO 4762 - Metric M4 x 25:1
- Mate:200: XEndStopHolder:1 ↔ BS EN ISO 4762 - Metric M4 x 25:1
- Mate:201: XEndStopHolder:1 ↔ BS EN ISO 4762 - Metric M4 x 25:2
- Mate:202: XEndStopHolder:1 ↔ BS EN ISO 4762 - Metric M4 x 25:2
- Mate:203: XEndStopHolder:1 ↔ BS EN ISO 4762 - Metric M4 x 25:3
- Mate:204: XEndStopHolder:1 ↔ BS EN ISO 4762 - Metric M4 x 25:3
- Mate:205: XEndStopHolder:1 ↔ BS EN ISO 4762 - Metric M4 x 25:4
- Mate:206: XEndStopHolder:1 ↔ BS EN ISO 4762 - Metric M4 x 25:4
- Mate:207: X Motor Bracket:1 ↔ XEndStopHolder:1
- Flush:51: Hotend:1 ↔ ISO 4026 M3 x 5:1
- Mate:208: E Motor Bracket:1 ↔ ISO 7380-1 M3 x 6:22
- Mate:209: Z Nut:1 ↔ ISO 7380-1 M3 x 6:22
- Mate:210: E Motor Bracket:1 ↔ ISO 7380-1 M3 x 6:23
- Mate:211: Z Nut:1 ↔ ISO 7380-1 M3 x 6:23
- Mate:212: Fan Cover:1 ↔ ISO 4762 M2 x 3:1
- Mate:213: Cold section fan:1 ↔ ISO 4762 M2 x 3:1
- Mate:218: Fan Cover:1 ↔ ISO 4762 M2 x 3:4
- Mate:219: Cold section fan:1 ↔ ISO 4762 M2 x 3:4
- Mate:220: Fan Cover:1 ↔ ISO 4762 M2 x 3:5
- Mate:221: Nozzle fan duct:1 ↔ ISO 4762 M2 x 3:5
- Mate:222: Fan Cover:1 ↔ ISO 4762 M2 x 3:6
- Mate:223: Nozzle fan duct:1 ↔ ISO 4762 M2 x 3:6
- Insert:65: Y Motor Bracket:1 ↔ ISO 7380-1 M3 x 16:2
- Insert:66: Y Motor Bracket:1 ↔ ISO 7380-1 M3 x 16:3
- Mate:224: Assembly1:5 ↔ ISO 7380-1 M3 x 8:1
- Mate:225: Y Motor Bracket:1 ↔ ISO 7380-1 M3 x 8:1
- Mate:226: Assembly1:5 ↔ ISO 7380-1 M3 x 8:2
- Mate:227: Y Motor Bracket:1 ↔ ISO 7380-1 M3 x 8:2
- Mate:228: Assembly1:5 ↔ ISO 7380-1 M3 x 8:3
- Mate:229: Y Motor Bracket:1 ↔ ISO 7380-1 M3 x 8:3
- Mate:230: Assembly1:5 ↔ ISO 7380-1 M3 x 8:4
- Mate:231: Y Motor Bracket:1 ↔ ISO 7380-1 M3 x 8:4
## Named parameters: d663_d661 = 0 mm
